# Autodesk Inventor assembly: main_assembly
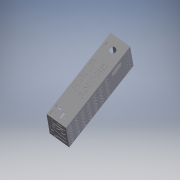
[picture p0: Inventor's stored thumbnail of the model, 180x180]
Saved by Autodesk Inventor 2016 (Build 200138000, 138)
## iProperties
Created: 2015-08-24
Part Number: main_assembly
Document SubType Name: Assembly
Designer: Chris Gerth
Author: Chris Gerth
## Documents named in this file (4)
- B:\Projects\RobotCasserole\RoboSim\enclosure2\main_assembly.iam
- B:\Projects\RobotCasserole\RoboSim\enclosure2\main_enclosure.ipt
- B:\Projects\RobotCasserole\RoboSim\enclosure2\arduino uno.iam
- B:\Projects\RobotCasserole\RoboSim\enclosure2\Fan 60x60x25mm.iam
## Components (3 placed, 3 different names)
1. main_enclosure:1 — Mate:1, Mate:2, Angle:1, Mate:3, Mate:4, Mate:5
2. arduino uno:1 [sub-assembly] — Mate:1, Mate:2, Angle:1
3. Fan 60x60x25mm:1 [sub-assembly] — Mate:3, Mate:4, Mate:5
## Relationships (6: Mate 5, Angle 1)
- Mate:1 (0.0508 mm): main_enclosure:1 ↔ arduino uno:1
- Mate:2: main_enclosure:1 ↔ arduino uno:1
- Angle:1 (0 deg): main_enclosure:1 ↔ arduino uno:1
- Mate:3: main_enclosure:1 ↔ Fan 60x60x25mm:1
- Mate:4 (25.4 mm): main_enclosure:1 ↔ Fan 60x60x25mm:1
- Mate:5 (57.15 mm): main_enclosure:1 ↔ Fan 60x60x25mm:1
